# Autodesk Inventor assembly: Gearbox with neverest
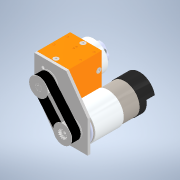
[picture p0: Inventor's stored thumbnail of the model, 180x180]
Saved by Autodesk Inventor 2020.2 (Build 242310000, 310)
## iProperties
Created: 2020-02-27
Part Number: Gearbox with neverest
Document SubType Name: Assembly
Designer: deli
Author: deli
## Documents named in this file (8)
- C:\Users\deli\OneDrive - Eastside Preparatory School\FTC\Chassi\Gearbox with neverest.iam
- C:\Users\deli\OneDrive - Eastside Preparatory School\FTC\Chassi\20-1 gearbox.iam
- C:\Users\deli\OneDrive - Eastside Preparatory School\FTC\Chassi\neveRest with 15T pinion.iam
- C:\Users\deli\OneDrive - Eastside Preparatory School\FTC\Chassi\.5 flanged bearing.ipt
- C:\Users\deli\OneDrive - Eastside Preparatory School\FTC\Chassi\Motor and gearbox panel.ipt
- C:\Users\deli\OneDrive - Eastside Preparatory School\FTC\Chassi\12T Pulley for neverest.ipt
- C:\Users\deli\OneDrive - Eastside Preparatory School\FTC\Chassi\12T Pulley for gearbox.ipt
- C:\Users\deli\OneDrive - Eastside Preparatory School\FTC\Chassi\43T timing belt from gobuilda.ipt
## Components (7 placed, 7 different names)
1. 20-1 gearbox:1 [sub-assembly] — Mate:1, Mate:2, Angle:1, Mate:14, Flush:2
2. .5 flanged bearing:1 — Mate:1, Mate:2
3. Motor and gearbox panel:1
4. neveRest with 15T pinion:1 [sub-assembly] — Flush:1, Mate:11, Mate:12
5. 12T Pulley for neverest:1 — Flush:1, Mate:11, Mate:12, Mate:16
6. 12T Pulley for gearbox:1 — Angle:1, Mate:14, Flush:2, Mate:15
7. 30T timing belt from westcoast products — Mate:15, Mate:16
## Relationships (10: Mate 7, Flush 2, Angle 1)
- Mate:1: 20-1 gearbox:1 ↔ .5 flanged bearing:1
- Mate:2: 20-1 gearbox:1 ↔ .5 flanged bearing:1
- Flush:1: neveRest with 15T pinion:1 ↔ 12T Pulley for neverest:1
- Mate:11: neveRest with 15T pinion:1 ↔ 12T Pulley for neverest:1
- Mate:12: neveRest with 15T pinion:1 ↔ 12T Pulley for neverest:1
- Angle:1 (0 deg): 20-1 gearbox:1 ↔ 12T Pulley for gearbox:1
- Mate:14: 20-1 gearbox:1 ↔ 12T Pulley for gearbox:1
- Flush:2: 20-1 gearbox:1 ↔ 12T Pulley for gearbox:1
- Mate:15: 12T Pulley for gearbox:1 ↔ 30T timing belt from westcoast products
- Mate:16: 12T Pulley for neverest:1 ↔ 30T timing belt from westcoast products
